# Autodesk Inventor assembly: SansCapacFata
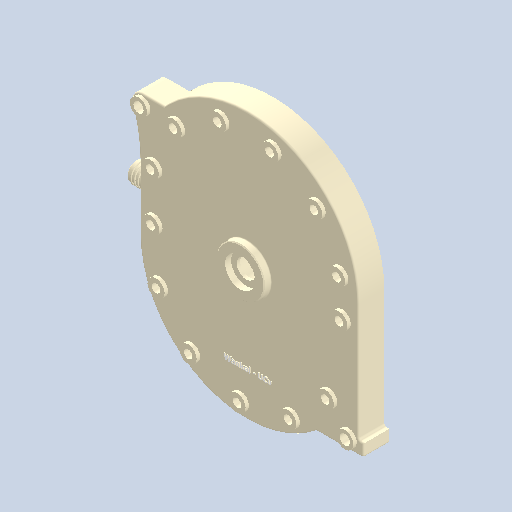
[picture p0: Inventor's stored thumbnail of the model, 512x512]
Saved by Autodesk Inventor 2022 (Build 260153000, 153)
## iProperties
Created: 2022-04-12
Part Number: SansCapacFata
Document SubType Name: Assembly
Designer: Janina
Author: Janina
## Documents named in this file (4)
- C:\Users\Janina\Desktop\CoceiJ\7 - Wankel\SansCapacFata.iam
- C:\Users\Janina\Desktop\CoceiJ\7 - Wankel\CapacFata.ipt
- C:\Users\Janina\Desktop\CoceiJ\7 - Wankel\Pinion.ipt
- C:\Users\Janina\Desktop\CoceiJ\7 - Wankel\SubansM4X10.iam
## Components (3 placed, 3 different names)
1. CapacFata:1 — Mate:1, Mate:2, Angle:1
2. Pinion:1 — Mate:1, Mate:2, Angle:1
3. SubansM4X10:1 [sub-assembly]
## Relationships (4: Mate 2, Angle 1, Insert 1)
- Mate:1: CapacFata:1 ↔ Pinion:1
- Mate:2: CapacFata:1 ↔ Pinion:1
- Angle:1 (99 deg): CapacFata:1 ↔ Pinion:1
- [Insert]: Pinion:1 ↔ SubansM4X10:1
